# Autodesk Inventor assembly: Rear_Wheel_Hub_Assembly
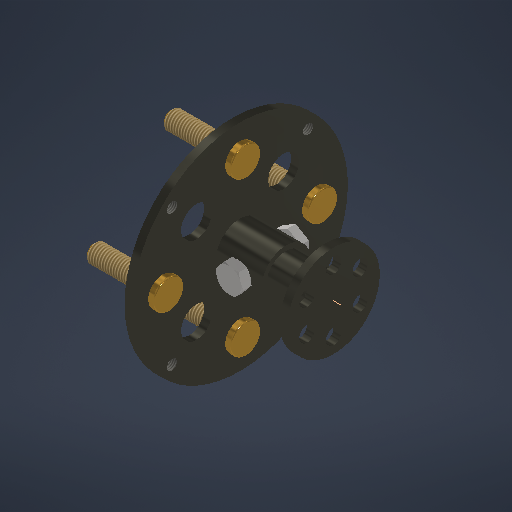
[picture p0: Inventor's stored thumbnail of the model, 512x512]
Saved by Autodesk Inventor 2026.1 (Build 301233000, 233)
## iProperties
Created: 2026-06-12
Part Number: Rear_Wheel_Hub_Assembly
Document SubType Name: Assembly
Designer: share
Author: share
## Documents named in this file (6)
- C:\Users\share\OneDrive\Documents\Personal Projects\GOGO Kart\CAD\GOGO_KART_FSAE\Drivetrain\Rear_Wheel_Hub_Assembly.iam
- C:\Users\share\OneDrive\Documents\Personal Projects\GOGO Kart\CAD\GOGO_KART_FSAE\Drivetrain\Hub-CV Adapter.ipt
- C:\Users\share\OneDrive\Documents\Personal Projects\GOGO Kart\CAD\GOGO_KART_FSAE\Drivetrain\Lug Stud M12 X 45.ipt
- C:\Users\share\OneDrive\Documents\Personal Projects\GOGO Kart\CAD\GOGO_KART_FSAE\Drivetrain\Hub.ipt
- C:\Users\share\OneDrive\Documents\Inventor\Content Center Files\R2026\en-US\AS 1110\AS 1110 - M10 x 40.ipt
- C:\Users\share\OneDrive\Documents\Inventor\Content Center Files\R2026\en-US\AS 1474(1)\AS 1474 - M10(1).ipt
## Components (8 placed, 5 different names)
1. Hub-CV Adapter:1 — Flush:1, Flush:2, Flush:3, Mate:1, Mate:2, Mate:5
2. Lug Stud M12 X 45:1 — Insert:2
3. Hub:1 — Mate:1, Mate:2, Insert:1, Insert:2, Insert:3, Insert:4, Mate:3, Mate:4
4. Lug Stud M12 X 45:2 — Insert:4
5. Lug Stud M12 X 45:3 — Insert:3
6. Lug Stud M12 X 45:4 — Insert:1
7. AS 1110 - Metric M10 x 40:1 — Mate:3, Mate:4, Flush:4
8. AS 1474 - Metric M10:1 — Mate:5, Flush:4
## Relationships (13: Mate 5, Flush 4, Insert 4)
- Flush:1: Hub-CV Adapter:1
- Flush:2: Hub-CV Adapter:1
- Flush:3: Hub-CV Adapter:1
- Mate:1: Hub-CV Adapter:1 ↔ Hub:1
- Mate:2: Hub-CV Adapter:1 ↔ Hub:1
- Insert:1: Hub:1 ↔ Lug Stud M12 X 45:4
- Insert:2: Lug Stud M12 X 45:1 ↔ Hub:1
- Insert:3: Hub:1 ↔ Lug Stud M12 X 45:3
- Insert:4: Hub:1 ↔ Lug Stud M12 X 45:2
- Mate:3: Hub:1 ↔ AS 1110 - Metric M10 x 40:1
- Mate:4: Hub:1 ↔ AS 1110 - Metric M10 x 40:1
- Mate:5: Hub-CV Adapter:1 ↔ AS 1474 - Metric M10:1
- Flush:4 (-3 mm): AS 1110 - Metric M10 x 40:1 ↔ AS 1474 - Metric M10:1
